# Autodesk Inventor assembly: Lacznik prosty sruby
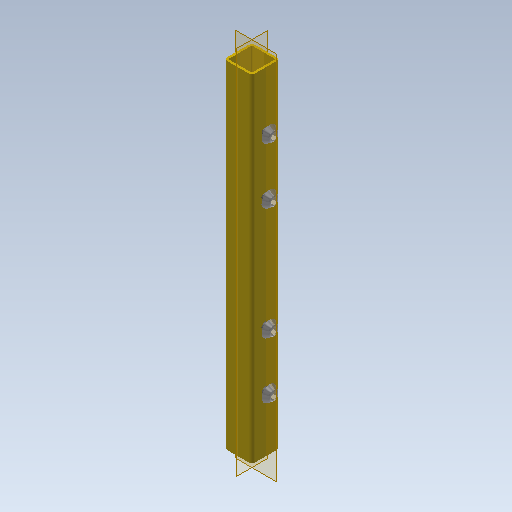
[picture p0: Inventor's stored thumbnail of the model, 512x512]
Saved by Autodesk Inventor 2021 (Build 250183000, 183)
## iProperties
Created: 2024-04-18
Part Number: Lacznik prosty sruby
Document SubType Name: Assembly
Designer: Michal
Author: Michal
## Documents named in this file (3)
- C:\Users\Michal\Documents\GitHub\PNW_PhotoBoothFrame_3D\Lacznik prosty sruby.iam
- C:\Users\Michal\Documents\GitHub\PNW_PhotoBoothFrame_3D\Lacznik prosty.ipt
- C:\Users\Michal\Documents\GitHub\PNW_PhotoBoothFrame_3D\M8x15.ipt
## Components (5 placed, 2 different names)
1. Lacznik prosty:1 — Mate:1, Mate:2, Mate:3, Mate:4, Mate:5
2. M8x15:1 — Mate:1, Flush:1, Flush:2, Flush:3, Mate:5
3. M8x15:2 — Mate:2, Flush:1
4. M8x15:3 — Mate:3, Flush:2
5. M8x15:4 — Mate:4, Flush:3
## Relationships (8: Mate 5, Flush 3)
- Mate:1: Lacznik prosty:1 ↔ M8x15:1
- Mate:2: Lacznik prosty:1 ↔ M8x15:2
- Mate:3: Lacznik prosty:1 ↔ M8x15:3
- Mate:4: Lacznik prosty:1 ↔ M8x15:4
- Flush:1: M8x15:1 ↔ M8x15:2
- Flush:2: M8x15:1 ↔ M8x15:3
- Flush:3: M8x15:1 ↔ M8x15:4
- Mate:5 (3 mm): Lacznik prosty:1 ↔ M8x15:1
